# Autodesk Inventor assembly: Pierna_opuesta
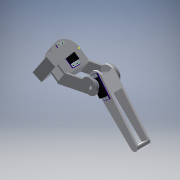
[picture p0: Inventor's stored thumbnail of the model, 180x180]
Saved by Autodesk Inventor 2018 (Build 220112000, 112)
## iProperties
Created: 2020-03-08
Part Number: Pierna_opuesta
Document SubType Name: Assembly
Designer: GonzaloDiaz
Author: GonzaloDiaz
## Documents named in this file (5)
- E:\Universidad\Codigo\Enigma\Diseños\Pierna_opuesta.iam
- E:\Universidad\Codigo\Enigma\Diseños\SERVOMG996R.ipt
- E:\Universidad\Codigo\Enigma\Diseños\Tibia_opuesta.ipt
- E:\Universidad\Codigo\Enigma\Diseños\Hombro.ipt
- E:\Universidad\Codigo\Enigma\Diseños\Femur.ipt
## Components (5 placed, 4 different names)
1. SERVOMG996R:1 — Mate:12, Mate:13, Mate:14
2. Tibia_opuesta:1 — Mate:9, Mate:10, Mate:11, Insert:1
3. SERVOMG996R:2 — Mate:9, Mate:10, Mate:11
4. Hombro:1 — Insert:2
5. Femur:1 — Insert:1, Mate:12, Mate:13, Mate:14, Insert:2
## Relationships (8: Mate 6, Insert 2)
- Mate:9: Tibia_opuesta:1 ↔ SERVOMG996R:2
- Mate:10: Tibia_opuesta:1 ↔ SERVOMG996R:2
- Mate:11: Tibia_opuesta:1 ↔ SERVOMG996R:2
- Insert:1: Tibia_opuesta:1 ↔ Femur:1
- Mate:12: SERVOMG996R:1 ↔ Femur:1
- Mate:13: SERVOMG996R:1 ↔ Femur:1
- Mate:14: SERVOMG996R:1 ↔ Femur:1
- Insert:2: Hombro:1 ↔ Femur:1
